# Autodesk Inventor assembly: V-Belt transmission4_MIR
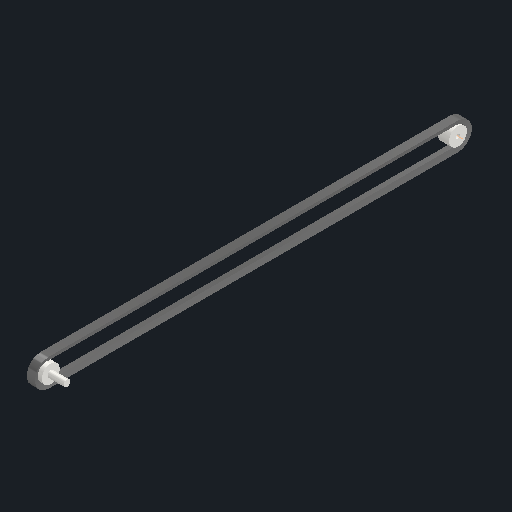
[picture p0: Inventor's stored thumbnail of the model, 512x512]
Saved by Autodesk Inventor 2024.2 (Build 282272000, 272)
## iProperties
Created: 2024-03-22
Part Number: V-Belt transmission4_MIR
Document SubType Name: Assembly
Designer: seifs
Author: LightStore
## Documents named in this file (4)
- C:\Users\seifs\Downloads\Final Assembly\V-Belt transmission4_MIR.iam
- C:\Users\seifs\Downloads\Final Assembly\V-Belt4_MIR.ipt
- C:\Users\seifs\Downloads\Final Assembly\Flat Pulley11_MIR.ipt
- C:\Users\seifs\Downloads\Final Assembly\Flat Pulley21_MIR.ipt
## Components (3 placed, 3 different names)
1. V-Belt4_MIR:1 — Mate:1, Flush:1, Mate:2, Flush:2
2. Flat Pulley11_MIR:1 — Mate:1, Flush:1, Rotation:1
3. Flat Pulley21_MIR:1 — Mate:2, Flush:2, Rotation:1
## Relationships (5: Mate 2, Flush 2, RelateRotation 1)
- Mate:1: V-Belt4_MIR:1 ↔ Flat Pulley11_MIR:1
- Flush:1: V-Belt4_MIR:1 ↔ Flat Pulley11_MIR:1
- Mate:2: V-Belt4_MIR:1 ↔ Flat Pulley21_MIR:1
- Flush:2: V-Belt4_MIR:1 ↔ Flat Pulley21_MIR:1
- Rotation:1 [RelateRotation] (1 ul): Flat Pulley11_MIR:1 ↔ Flat Pulley21_MIR:1
